# Autodesk Inventor assembly: HTD-45H
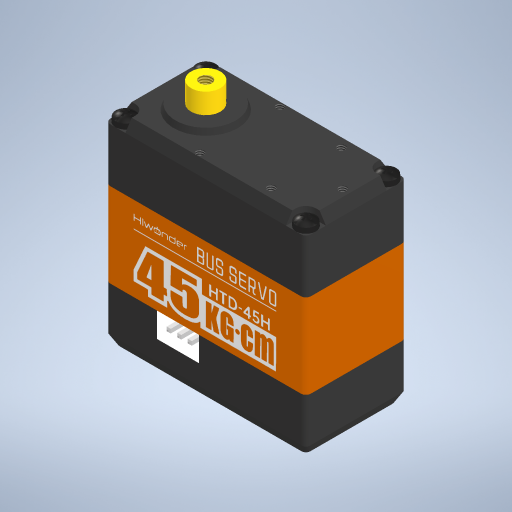
[picture p0: Inventor's stored thumbnail of the model, 512x512]
Saved by Autodesk Inventor 2024.1 (Build 281209000, 209)
## iProperties
Created: 2023-08-18
Part Number: HTD-45H
Document SubType Name: Assembly
Designer: chanh
Author: chanh
## Documents named in this file (3)
- C:\Users\chanh\OneDrive - 연세대학교 (Yonsei University)\로봇\Humanoid\Roboin Humanoid Project\Roboin Humanoid Project [Part5]\HTD-45H, Horn\HTD-45H\HTD-45H.iam
- C:\Users\chanh\OneDrive - 연세대학교 (Yonsei University)\로봇\Humanoid\Roboin Humanoid Project\Roboin Humanoid Project [Part5]\HTD-45H, Horn\HTD-45H\HTD-45H.ipt
- C:\Users\chanh\OneDrive - 연세대학교 (Yonsei University)\로봇\Humanoid\Roboin Humanoid Project\Roboin Humanoid Project [Part5]\HTD-45H, Horn\HTD-45H\M2x32.ipt
## Components (5 placed, 2 different names)
1. HTD-45H:1 — Flush:1, Flush:2, Flush:3, Rigid:1, Rigid:2, Rigid:3, Rigid:4
2. M2x32:1 — Rigid:1
3. M2x32:2 — Rigid:2
4. M2x32:3 — Rigid:3
5. M2x32:4 — Rigid:4
## Relationships (7: WeldJoint 4, Flush 3)
- Flush:1: HTD-45H:1
- Flush:2: HTD-45H:1
- Flush:3: HTD-45H:1
- Rigid:1 [WeldJoint]: HTD-45H:1 ↔ M2x32:1
- Rigid:2 [WeldJoint]: HTD-45H:1 ↔ M2x32:2
- Rigid:3 [WeldJoint]: HTD-45H:1 ↔ M2x32:3
- Rigid:4 [WeldJoint]: HTD-45H:1 ↔ M2x32:4
